# Autodesk Inventor assembly: 상단 조립품
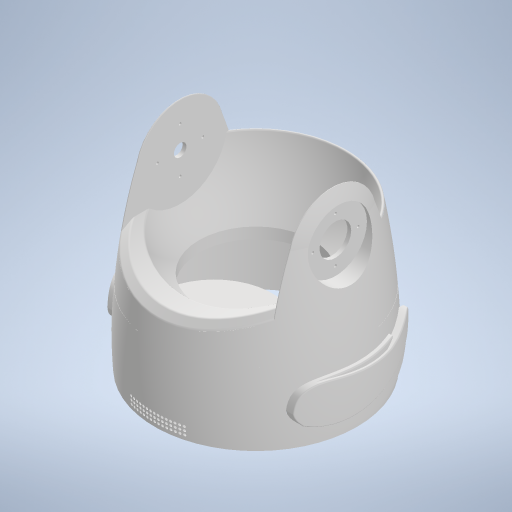
[picture p0: Inventor's stored thumbnail of the model, 512x512]
Saved by Autodesk Inventor 2023 (Build 270158000, 158)
## iProperties
Created: 2022-08-14
Part Number: 상단 조립품
Document SubType Name: Assembly
Designer: fly01
Author: fly01
## Documents named in this file (6)
- C:\Users\user\Desktop\PAI\PAI설계\조림품\상단 조립품.iam
- C:\Users\user\Desktop\PAI\PAI설계\범용 부품\스피커.ipt
- C:\Users\user\Desktop\PAI\PAI설계\출력품\상단 서보모터 고정 판.ipt
- C:\Users\user\Desktop\PAI\PAI설계\범용 부품\십자 둥근머리 볼트 M2 10mm.ipt
- C:\Users\user\Desktop\PAI\PAI설계\출력품\body_top_2.ipt
- C:\Users\user\Desktop\PAI\PAI설계\출력품\body_top1.ipt
## Components (6 placed, 5 different names)
1. 스피커:1 — 삽입:13
2. 상단 서보모터 고정 판:1 — 삽입:6, 삽입:7, 삽입:14, 삽입:15
3. 십자 둥근머리 볼트 M2 10mm:1 — 삽입:6
4. 십자 둥근머리 볼트 M2 10mm:2 — 삽입:7
5. body_top_2:1 — 삽입:8, 삽입:9, 삽입:13, 삽입:14, 삽입:15
6. body_top1:1 — 삽입:8, 삽입:9
## Relationships (7: Insert 7)
- 삽입:6 [Insert]: 상단 서보모터 고정 판:1 ↔ 십자 둥근머리 볼트 M2 10mm:1
- 삽입:7 [Insert]: 상단 서보모터 고정 판:1 ↔ 십자 둥근머리 볼트 M2 10mm:2
- 삽입:8 [Insert]: body_top_2:1 ↔ body_top1:1
- 삽입:9 [Insert]: body_top_2:1 ↔ body_top1:1
- 삽입:13 [Insert]: 스피커:1 ↔ body_top_2:1
- 삽입:14 [Insert]: 상단 서보모터 고정 판:1 ↔ body_top_2:1
- 삽입:15 [Insert]: 상단 서보모터 고정 판:1 ↔ body_top_2:1
